# Autodesk Inventor assembly: V-Belt transmission
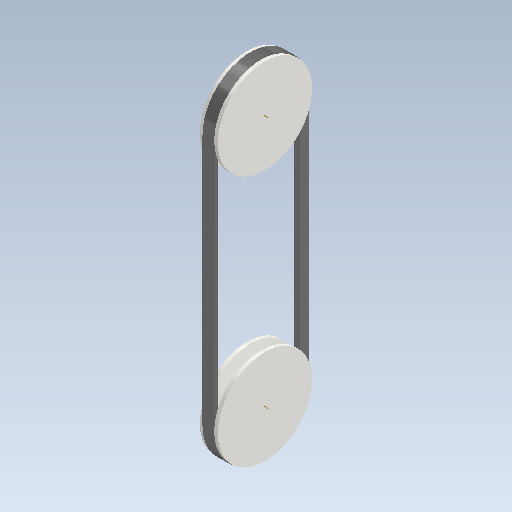
[picture p0: Inventor's stored thumbnail of the model, 512x512]
Saved by Autodesk Inventor 2021 (Build 250183000, 183)
## iProperties
ClientObjectVersion: 1
Created: 2021-04-20
Part Number: V-Belt transmission
Document SubType Name: Assembly
Designer: calst
Author: calst
## Documents named in this file (4)
- C:\Users\calst\OneDrive\Desktop\University Work\Year 3\Semester 2\Integrated Group Robotics Project\Group Task\AutoDesk Inventor\Final Parts\bELT\Design Accelerator\V-Belt transmission1.iam
- C:\Users\calst\OneDrive\Desktop\University Work\Year 3\Semester 2\Integrated Group Robotics Project\Group Task\AutoDesk Inventor\Final Parts\bELT\Design Accelerator\V-Belt1.ipt
- C:\Users\calst\OneDrive\Desktop\University Work\Year 3\Semester 2\Integrated Group Robotics Project\Group Task\AutoDesk Inventor\Final Parts\bELT\Design Accelerator\Grooved Pulley11.ipt
- C:\Users\calst\OneDrive\Desktop\University Work\Year 3\Semester 2\Integrated Group Robotics Project\Group Task\AutoDesk Inventor\Final Parts\bELT\Design Accelerator\Grooved Pulley21.ipt
## Components (3 placed, 3 different names)
1. Grooved Pulley1:1 — Flush:1, Mate:1, Rotation:1
2. Grooved Pulley2:1 — Flush:2, Mate:2, Rotation:1
3. V-Belt:1 — Flush:1, Mate:1, Flush:2, Mate:2
## Component patterns: (1 elements, first: V-Belt:1)
## Relationships (5: Flush 2, Mate 2, RelateRotation 1)
- Flush:1: Grooved Pulley1:1 ↔ V-Belt:1
- Mate:1: Grooved Pulley1:1 ↔ V-Belt:1
- Flush:2: Grooved Pulley2:1 ↔ V-Belt:1
- Mate:2: Grooved Pulley2:1 ↔ V-Belt:1
- Rotation:1 [RelateRotation] (1 ul): Grooved Pulley1:1 ↔ Grooved Pulley2:1
